# Autodesk Inventor assembly: final_assembly
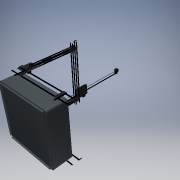
[picture p0: Inventor's stored thumbnail of the model, 180x180]
Saved by Autodesk Inventor 2018 (Build 220112000, 112)
## iProperties
Created: 2017-11-25
Part Number: final_assembly
Document SubType Name: Assembly
Designer: g
Author: g
## Documents named in this file (5)
- C:\Users\g\Desktop\AUG_inventor\final_assembly.iam
- C:\Users\g\Desktop\AUG_inventor\base_assembly.iam
- C:\Users\g\Desktop\AUG_inventor\gantry_assembly.iam
- C:\Users\g\Desktop\AUG_inventor\z_carriage_assembly.iam
- C:\Users\g\Desktop\AUG_inventor\y_carriage_assembly.iam
## Components (4 placed, 4 different names)
1. base_assembly:1 [sub-assembly] — Mate:1, Tangent:2, Tangent:6, Flush:1
2. gantry_assembly:1 [sub-assembly] — Mate:1, Tangent:2, Tangent:6, Mate:5, Tangent:8, Tangent:9, Flush:1, Mate:7, Tangent:11
3. z_carriage_assembly:1 [sub-assembly] — Mate:5, Tangent:8, Tangent:9, Mate:6, Tangent:10, Tangent:11
4. y_carriage_assembly:1 [sub-assembly] — Mate:6, Tangent:10, Mate:7
## Relationships (11: Tangent 6, Mate 4, Flush 1)
- Mate:1: base_assembly:1 ↔ gantry_assembly:1
- Tangent:2: base_assembly:1 ↔ gantry_assembly:1
- Tangent:6: base_assembly:1 ↔ gantry_assembly:1
- Mate:5: gantry_assembly:1 ↔ z_carriage_assembly:1
- Tangent:8: gantry_assembly:1 ↔ z_carriage_assembly:1
- Tangent:9: gantry_assembly:1 ↔ z_carriage_assembly:1
- Mate:6: z_carriage_assembly:1 ↔ y_carriage_assembly:1
- Tangent:10: z_carriage_assembly:1 ↔ y_carriage_assembly:1
- Flush:1: base_assembly:1 ↔ gantry_assembly:1
- Mate:7: gantry_assembly:1 ↔ y_carriage_assembly:1
- Tangent:11: gantry_assembly:1 ↔ z_carriage_assembly:1
